# Autodesk Inventor assembly: mainboard 1
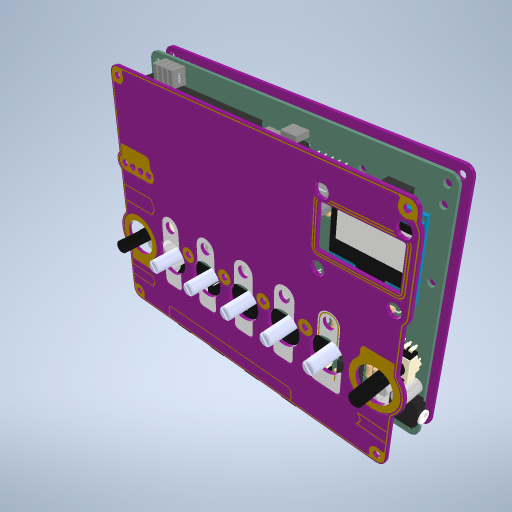
[picture p0: Inventor's stored thumbnail of the model, 512x512]
Saved by Autodesk Inventor 2024 (Build 280153000, 153)
## iProperties
Company: Kicad
Created: 2023-11-29
Part Number: mainboard 1
Description: KiCad electronic assembly
Document SubType Name: Assembly
Designer: Ishaan
Authority: Unknown
Sending System: KiCad to STEP converter
Preprocessor: Open CASCADE STEP processor 7.6
Title: mainboard.step
Author: Pcbnew
## Documents named in this file (21)
- D:\Dropbox (MIT)\Dropbox (MIT)\School Related\IAP DSP COURSE\Foxglove-DSP-Amplifier\Amplifier MCAD\mainboard\mainboard.iam
- D:\Dropbox (MIT)\Dropbox (MIT)\School Related\IAP DSP COURSE\Foxglove-DSP-Amplifier\Amplifier MCAD\mainboard\WURTH_860020x730xx.iam
- D:\Dropbox (MIT)\Dropbox (MIT)\School Related\IAP DSP COURSE\Foxglove-DSP-Amplifier\Amplifier MCAD\mainboard\R82EC2100AA50J.iam
- D:\Dropbox (MIT)\Dropbox (MIT)\School Related\IAP DSP COURSE\Foxglove-DSP-Amplifier\Amplifier MCAD\mainboard\R_Axial_DIN0207_L6.3mm_D2.5mm_P10.16mm_Horizontal.iam
- D:\Dropbox (MIT)\Dropbox (MIT)\School Related\IAP DSP COURSE\Foxglove-DSP-Amplifier\Amplifier MCAD\mainboard\EC11-THT-25R-black.iam
- D:\Dropbox (MIT)\Dropbox (MIT)\School Related\IAP DSP COURSE\Foxglove-DSP-Amplifier\Amplifier MCAD\mainboard\SH1106_LCD_1.3.iam
- D:\Dropbox (MIT)\Dropbox (MIT)\School Related\IAP DSP COURSE\Foxglove-DSP-Amplifier\Amplifier MCAD\mainboard\PinSocket_1x04_P2.54mm_Vertical.iam
- D:\Dropbox (MIT)\Dropbox (MIT)\School Related\IAP DSP COURSE\Foxglove-DSP-Amplifier\Amplifier MCAD\mainboard\PinHeader_1x04_P2.54mm_Vertical.iam
- D:\Dropbox (MIT)\Dropbox (MIT)\School Related\IAP DSP COURSE\Foxglove-DSP-Amplifier\Amplifier MCAD\mainboard\LED_D5.0mm-4_RGB.iam
- D:\Dropbox (MIT)\Dropbox (MIT)\School Related\IAP DSP COURSE\Foxglove-DSP-Amplifier\Amplifier MCAD\mainboard\nmj6hfd2.iam
- D:\Dropbox (MIT)\Dropbox (MIT)\School Related\IAP DSP COURSE\Foxglove-DSP-Amplifier\Amplifier MCAD\mainboard\LED_D3.0mm_Clear.iam
- D:\Dropbox (MIT)\Dropbox (MIT)\School Related\IAP DSP COURSE\Foxglove-DSP-Amplifier\Amplifier MCAD\mainboard\PinSocket_1x24_P2.54mm_Vertical.iam
- D:\Dropbox (MIT)\Dropbox (MIT)\School Related\IAP DSP COURSE\Foxglove-DSP-Amplifier\Amplifier MCAD\mainboard\PinHeader_1x24_P2.54mm_Vertical.iam
- D:\Dropbox (MIT)\Dropbox (MIT)\School Related\IAP DSP COURSE\Foxglove-DSP-Amplifier\Amplifier MCAD\mainboard\Teensy 4.1.iam
- D:\Dropbox (MIT)\Dropbox (MIT)\School Related\IAP DSP COURSE\Foxglove-DSP-Amplifier\Amplifier MCAD\mainboard\DIP-14_W7.62mm_Socket.iam
- D:\Dropbox (MIT)\Dropbox (MIT)\School Related\IAP DSP COURSE\Foxglove-DSP-Amplifier\Amplifier MCAD\mainboard\DIP-14_W7.62mm.iam
- D:\Dropbox (MIT)\Dropbox (MIT)\School Related\IAP DSP COURSE\Foxglove-DSP-Amplifier\Amplifier MCAD\mainboard\ptv09a-4x30u-xxxx.iam
- D:\Dropbox (MIT)\Dropbox (MIT)\School Related\IAP DSP COURSE\Foxglove-DSP-Amplifier\Amplifier MCAD\mainboard\pj-307.iam
- D:\Dropbox (MIT)\Dropbox (MIT)\School Related\IAP DSP COURSE\Foxglove-DSP-Amplifier\Amplifier MCAD\mainboard\Amplifier Hardware R1 PCB.ipt
- D:\Dropbox (MIT)\Dropbox (MIT)\School Related\IAP DSP COURSE\Foxglove-DSP-Amplifier\Amplifier MCAD\top_cover\top_cover_template.ipt
- D:\Dropbox (MIT)\Dropbox (MIT)\School Related\IAP DSP COURSE\Foxglove-DSP-Amplifier\Amplifier MCAD\bot_cover\bot_cover_template.ipt
## Components (126 placed, 126 different names)
1. 2 [sub-assembly]
2. 4 [sub-assembly]
3. 6 [sub-assembly]
4. 7 [sub-assembly]
5. 8 [sub-assembly]
6. 9 [sub-assembly]
7. 10 [sub-assembly]
8. 11 [sub-assembly]
9. 13 [sub-assembly]
10. 14 [sub-assembly]
11. 15 [sub-assembly]
12. 16 [sub-assembly]
13. 17 [sub-assembly]
14. 19 [sub-assembly]
15. 21 [sub-assembly]
16. 23 [sub-assembly]
17. 25 [sub-assembly]
18. 26 [sub-assembly]
19. 27 [sub-assembly]
20. 28 [sub-assembly]
21. 29 [sub-assembly]
22. 30 [sub-assembly]
23. 32 [sub-assembly]
24. 33 [sub-assembly]
25. 34 [sub-assembly]
26. 35 [sub-assembly]
27. 36 [sub-assembly]
28. 37 [sub-assembly]
29. 38 [sub-assembly]
30. 39 [sub-assembly]
31. 40 [sub-assembly]
32. 41 [sub-assembly]
33. 42 [sub-assembly]
34. 43 [sub-assembly]
35. 44 [sub-assembly]
36. 45 [sub-assembly]
37. 46 [sub-assembly]
38. 47 [sub-assembly]
39. 48 [sub-assembly]
40. 49 [sub-assembly]
41. 50 [sub-assembly]
42. 51 [sub-assembly]
43. 52 [sub-assembly]
44. 53 [sub-assembly]
45. 54 [sub-assembly]
46. 55 [sub-assembly]
47. 56 [sub-assembly]
48. 57 [sub-assembly]
49. 59 [sub-assembly]
50. 60 [sub-assembly]
51. 61 [sub-assembly]
52. 62 [sub-assembly]
53. 64 [sub-assembly]
54. 65 [sub-assembly]
55. 67 [sub-assembly]
56. 68 [sub-assembly]
57. 70 [sub-assembly]
58. 71 [sub-assembly]
59. 72 [sub-assembly]
60. 73 [sub-assembly]
61. 74 [sub-assembly]
62. 75 [sub-assembly]
63. 77 [sub-assembly]
64. 79 [sub-assembly]
65. 80 [sub-assembly]
66. 81 [sub-assembly]
67. 82 [sub-assembly]
68. 83 [sub-assembly]
69. 84 [sub-assembly]
70. 85 [sub-assembly]
71. 86 [sub-assembly]
72. 87 [sub-assembly]
73. 88 [sub-assembly]
74. 89 [sub-assembly]
75. 90 [sub-assembly]
76. 91 [sub-assembly]
77. 92 [sub-assembly]
78. 93 [sub-assembly]
79. 94 [sub-assembly]
80. 95 [sub-assembly]
81. 96 [sub-assembly]
82. 97 [sub-assembly]
83. 98 [sub-assembly]
84. 99 [sub-assembly]
85. 100 [sub-assembly]
86. 102 [sub-assembly]
87. 103 [sub-assembly]
88. 104 [sub-assembly]
89. 105 [sub-assembly]
90. 106 [sub-assembly]
91. 107 [sub-assembly]
92. 108 [sub-assembly]
93. 109 [sub-assembly]
94. 111 [sub-assembly]
95. 112 [sub-assembly]
96. 113 [sub-assembly]
97. 114 [sub-assembly]
98. 115 [sub-assembly]
99. 116 [sub-assembly]
100. 117 [sub-assembly]
101. 118 [sub-assembly]
102. 119 [sub-assembly]
103. 120 [sub-assembly]
104. 121 [sub-assembly]
105. 122 [sub-assembly]
106. 123 [sub-assembly]
107. 124 [sub-assembly]
108. 125 [sub-assembly]
109. 126 [sub-assembly]
110. 127 [sub-assembly]
111. 128 [sub-assembly]
112. 129 [sub-assembly]
113. 130 [sub-assembly]
114. 131 [sub-assembly]
115. 132 [sub-assembly]
116. 133 [sub-assembly]
117. 134 [sub-assembly]
118. 135 [sub-assembly]
119. 136 [sub-assembly]
120. 137 [sub-assembly]
121. 138 [sub-assembly]
122. 139 [sub-assembly]
123. 140 [sub-assembly]
124. 141 — Mate:1, Mate:2, Mate:3, Insert:1, Insert:2
125. top_cover_template:1 — Mate:1, Mate:2, Mate:3
126. bot_cover_template:1 — Insert:1, Insert:2
## Relationships (5: Mate 3, Insert 2)
- Mate:1: 141 ↔ top_cover_template:1
- Mate:2: 141 ↔ top_cover_template:1
- Mate:3 (18 mm): 141 ↔ top_cover_template:1
- Insert:1 (6 mm): 141 ↔ bot_cover_template:1
- Insert:2 (6 mm): 141 ↔ bot_cover_template:1
